# Autodesk Inventor assembly: NASA-20-FR
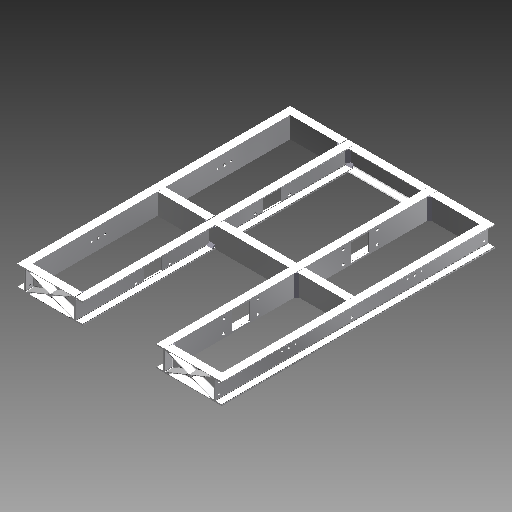
[picture p0: Inventor's stored thumbnail of the model, 512x512]
Saved by Autodesk Inventor 2020 (Build 240168000, 168)
## iProperties
Created: 2019-09-07
Part Number: NASA-20-FR
Document SubType Name: Weldment
Designer: Rick Szalay
Weld Material: Welded Aluminum-6061
Mass: 2639.52 g
Surface Area: 6820.5 cm^2
Volume: 977.588 cm^3
Density: 2.70004 g/cm^3
Author: Rick Szalay
## Documents named in this file (7)
- C:\Users\Matt\OneDrive\Inventor\NASA 2020\NASA 20\NASA-20\NASA-20\FR\NASA-20-FR.iam
- C:\Users\Matt\OneDrive\Inventor\NASA 2020\NASA 20\NASA-20\NASA-20\FR\NASA-20-FR-SP-01.ipt
- C:\Users\Matt\OneDrive\Inventor\NASA 2020\NASA 20\NASA-20\NASA-20\FR\NASA-20-FR-BK-01.ipt
- C:\Users\Matt\OneDrive\Inventor\NASA 2020\NASA 20\NASA-20\NASA-20\FR\NASA-20-FR-FP-01.ipt
- C:\Users\Matt\OneDrive\Inventor\NASA 2020\NASA 20\NASA-20\NASA-20\FR\NASA-20-FR-TB-01.ipt
- C:\Users\Matt\OneDrive\Inventor\NASA 2020\NASA 20\NASA-20\NASA-20\FR\NASA-20-FR-OP-01.ipt
- C:\Users\Rick Szalay\Documents\Inventor\Content Center Files\R2020\en-US\ANSI B18.3(05)\ANSI B18.3 - 10-24 UNC - 0.375(31).ipt
## Components (24 placed, 6 different names)
1. NASA-20-FR-TB-01:1
2. NASA-20-FR-TB-01:2
3. NASA-20-FR-TB-01:3 — Flush:19
4. NASA-20-FR-TB-01:4
5. NASA-20-FR-TB-01:5 — Flush:18
6. NASA-20-FR-TB-01:6
7. NASA-20-FR-SP-01:1 — Mate:3, Mate:4
8. NASA-20-FR-SP-01:2 — Mate:3
9. NASA-20-FR-BK-01:1 — Flush:7, Mate:5
10. NASA-20-FR-FP-01:1 — Mate:5, Flush:18, Flush:19
11. NASA-20-FR-OP-01:2 — Insert:7, Insert:8, Insert:9, Insert:10, Insert:11, Insert:12
12. NASA-20-FR-OP-01:1 — Insert:1, Insert:2, Insert:3, Insert:4, Insert:5, Insert:6
13. Hexagon Socket Head Cap Screw - Inch No. 10 - 24 UNC - 3/8:2 — Insert:1
14. Hexagon Socket Head Cap Screw - Inch No. 10 - 24 UNC - 3/8:3 — Insert:2
15. Hexagon Socket Head Cap Screw - Inch No. 10 - 24 UNC - 3/8:4 — Insert:3
16. Hexagon Socket Head Cap Screw - Inch No. 10 - 24 UNC - 3/8:5 — Insert:4
17. Hexagon Socket Head Cap Screw - Inch No. 10 - 24 UNC - 3/8:6 — Insert:5
18. Hexagon Socket Head Cap Screw - Inch No. 10 - 24 UNC - 3/8:7 — Insert:6
19. Hexagon Socket Head Cap Screw - Inch No. 10 - 24 UNC - 3/8:8 — Insert:7
20. Hexagon Socket Head Cap Screw - Inch No. 10 - 24 UNC - 3/8:9 — Insert:8
21. Hexagon Socket Head Cap Screw - Inch No. 10 - 24 UNC - 3/8:10 — Insert:9
22. Hexagon Socket Head Cap Screw - Inch No. 10 - 24 UNC - 3/8:1 — Insert:10
23. Hexagon Socket Head Cap Screw - Inch No. 10 - 24 UNC - 3/8:11 — Insert:11
24. Hexagon Socket Head Cap Screw - Inch No. 10 - 24 UNC - 3/8:12 — Insert:12
## Relationships (47: Flush 22, Mate 13, Insert 12)
- [Flush]: NASA-20-FR-SP-01:1 ↔ NASA-20-FR-SP-01:2
- [Flush]: NASA-20-FR-SP-01:1 ↔ NASA-20-FR-SP-01:2
- [Flush]: NASA-20-FR-SP-01:1 ↔ NASA-20-FR-BK-01:1
- [Flush]: NASA-20-FR-SP-01:1 ↔ NASA-20-FR-BK-01:1
- [Mate]: NASA-20-FR-SP-01:1 ↔ NASA-20-FR-BK-01:1
- [Mate]: NASA-20-FR-SP-01:1 ↔ NASA-20-FR-FP-01:1
- [Flush]: NASA-20-FR-SP-01:1 ↔ NASA-20-FR-FP-01:1
- Mate:3 (-215.9 mm): NASA-20-FR-SP-01:1 ↔ NASA-20-FR-SP-01:2
- Mate:4: NASA-20-FR-SP-01:1
- Flush:7: NASA-20-FR-BK-01:1
- Mate:5 (-339.725 mm): NASA-20-FR-BK-01:1 ↔ NASA-20-FR-FP-01:1
- [Mate]: NASA-20-FR-TB-01:1 ↔ NASA-20-FR-SP-01:2
- [Flush]: NASA-20-FR-TB-01:1 ↔ NASA-20-FR-BK-01:1
- [Flush]: NASA-20-FR-TB-01:1 ↔ NASA-20-FR-SP-01:2
- [Mate]: NASA-20-FR-TB-01:3 ↔ NASA-20-FR-SP-01:2
- [Flush]: NASA-20-FR-TB-01:3 ↔ NASA-20-FR-SP-01:2
- [Mate]: NASA-20-FR-TB-01:2 ↔ NASA-20-FR-SP-01:2
- [Flush]: NASA-20-FR-TB-01:2 ↔ NASA-20-FR-SP-01:2
- [Flush]: NASA-20-FR-TB-01:2 ↔ NASA-20-FR-SP-01:2
- [Mate]: NASA-20-FR-TB-01:6 ↔ NASA-20-FR-SP-01:1
- [Mate]: NASA-20-FR-TB-01:5 ↔ NASA-20-FR-SP-01:1
- [Mate]: NASA-20-FR-TB-01:4 ↔ NASA-20-FR-SP-01:1
- [Flush]: NASA-20-FR-TB-01:5 ↔ NASA-20-FR-SP-01:1
- [Flush]: NASA-20-FR-TB-01:6 ↔ NASA-20-FR-BK-01:1
- [Flush]: NASA-20-FR-TB-01:4 ↔ NASA-20-FR-SP-01:1
- [Flush]: NASA-20-FR-TB-01:4 ↔ NASA-20-FR-SP-01:1
- [Flush]: NASA-20-FR-TB-01:6 ↔ NASA-20-FR-BK-01:1
- Flush:18: NASA-20-FR-TB-01:5 ↔ NASA-20-FR-FP-01:1
- Flush:19: NASA-20-FR-TB-01:3 ↔ NASA-20-FR-FP-01:1
- [Flush]: NASA-20-FR-OP-01:2 ↔ NASA-20-FR-OP-01:1
- [Flush]: NASA-20-FR-OP-01:2 ↔ NASA-20-FR-OP-01:1
- [Flush]: NASA-20-FR-SP-01:1 ↔ NASA-20-FR-OP-01:1
- [Flush]: NASA-20-FR-SP-01:1 ↔ NASA-20-FR-OP-01:1
- [Mate]: NASA-20-FR-TB-01:3 ↔ NASA-20-FR-OP-01:2
- [Mate]: NASA-20-FR-TB-01:5 ↔ NASA-20-FR-OP-01:1
- Insert:1: NASA-20-FR-OP-01:1 ↔ Hexagon Socket Head Cap Screw - Inch No. 10 - 24 UNC - 3/8:2
- Insert:2: NASA-20-FR-OP-01:1 ↔ Hexagon Socket Head Cap Screw - Inch No. 10 - 24 UNC - 3/8:3
- Insert:3: NASA-20-FR-OP-01:1 ↔ Hexagon Socket Head Cap Screw - Inch No. 10 - 24 UNC - 3/8:4
- Insert:4: NASA-20-FR-OP-01:1 ↔ Hexagon Socket Head Cap Screw - Inch No. 10 - 24 UNC - 3/8:5
- Insert:5: NASA-20-FR-OP-01:1 ↔ Hexagon Socket Head Cap Screw - Inch No. 10 - 24 UNC - 3/8:6
- Insert:6: NASA-20-FR-OP-01:1 ↔ Hexagon Socket Head Cap Screw - Inch No. 10 - 24 UNC - 3/8:7
- Insert:7: NASA-20-FR-OP-01:2 ↔ Hexagon Socket Head Cap Screw - Inch No. 10 - 24 UNC - 3/8:8
- Insert:8: NASA-20-FR-OP-01:2 ↔ Hexagon Socket Head Cap Screw - Inch No. 10 - 24 UNC - 3/8:9
- Insert:9: NASA-20-FR-OP-01:2 ↔ Hexagon Socket Head Cap Screw - Inch No. 10 - 24 UNC - 3/8:10
- Insert:10: NASA-20-FR-OP-01:2 ↔ Hexagon Socket Head Cap Screw - Inch No. 10 - 24 UNC - 3/8:1
- Insert:11: NASA-20-FR-OP-01:2 ↔ Hexagon Socket Head Cap Screw - Inch No. 10 - 24 UNC - 3/8:11
- Insert:12: NASA-20-FR-OP-01:2 ↔ Hexagon Socket Head Cap Screw - Inch No. 10 - 24 UNC - 3/8:12
## Named parameters: Width = 215.9 mm, Length = 660.4 mm
